# Autodesk Inventor assembly: GearV1
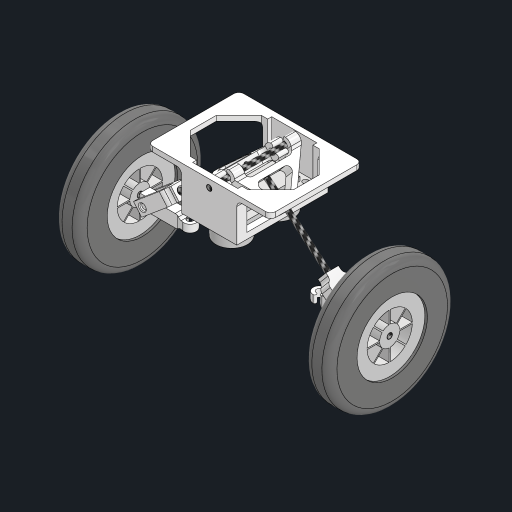
[picture p0: Inventor's stored thumbnail of the model, 512x512]
Saved by Autodesk Inventor 2023 (Build 270158000, 158)
## iProperties
Created: 2022-06-24
Part Number: GearV1
Document SubType Name: Assembly
Designer: legot
Author: legot
## Documents named in this file (11)
- C:\Users\legot\Documents\Inventor\HIKOSAPO\Gear\GearV1.iam
- C:\Users\legot\Documents\Inventor\HIKOSAPO\Ultrasonic_holderV4.ipt
- C:\Users\legot\Documents\Inventor\HIKOSAPO\Gear\Holder's Shaft.ipt
- C:\Users\legot\Documents\Inventor\HIKOSAPO\Gear\GearBase.ipt
- C:\Users\legot\Documents\Inventor\HIKOSAPO\UltrasonicSensor.ipt
- C:\Users\legot\Documents\Inventor\HIKOSAPO\Gear\gear_rod.ipt
- C:\Users\legot\Documents\Inventor\HIKOSAPO\Gear\gear_connecotr1.ipt
- C:\Users\legot\Documents\Inventor\HIKOSAPO\Gear\gear_connector2.ipt
- C:\Users\legot\Documents\Inventor\HIKOSAPO\Gear\gear_shaft1.ipt
- C:\Users\legot\Documents\Inventor\HIKOSAPO\Gear\Tire_Φ50.ipt
- C:\Users\legot\Documents\Inventor\HIKOSAPO\Gear\Wheel_Φ50.ipt
## Components (17 placed, 10 different names)
1. Ultrasonic_holderV4:1 — 挿入:4, 挿入:5, 角度:2, 挿入:14, 挿入:15, 挿入:16, 角度:3
2. Holder's Shaft:1 — 挿入:14
3. GearBase:1 — 挿入:6, 挿入:16, 角度:3
4. GearBase:2 — 挿入:7, 角度:2, 挿入:15
5. UltrasonicSensor:1 — 挿入:4, 挿入:5
6. gear_rod:1 — 挿入:6, 挿入:8
7. gear_rod:2 — 挿入:7, 挿入:9
8. gear_connecotr1:1 — メイト:1, メイト:4, フラッシュ:1, 挿入:10
9. gear_connecotr1:2 — メイト:2, メイト:3, フラッシュ:1, 挿入:11
10. gear_connector2:1 — 挿入:8, メイト:1, メイト:4
11. gear_connector2:2 — 挿入:9, メイト:2, メイト:3
12. gear_shaft1:1 — 挿入:11, 挿入:18
13. gear_shaft1:2 — 挿入:10, 挿入:17
14. Tire_Φ50:1 — フラッシュ:2, メイト:5
15. Tire_Φ50:2 — フラッシュ:3, メイト:6
16. Wheel_Φ50:1 — フラッシュ:2, メイト:5, 挿入:17
17. Wheel_Φ50:2 — フラッシュ:3, 挿入:18, メイト:6
## Relationships (24: Insert 13, Mate 6, Flush 3, Angle 2)
- 挿入:4 [Insert]: Ultrasonic_holderV4:1 ↔ UltrasonicSensor:1
- 挿入:5 [Insert]: Ultrasonic_holderV4:1 ↔ UltrasonicSensor:1
- 挿入:6 [Insert]: GearBase:1 ↔ gear_rod:1
- 挿入:7 [Insert]: GearBase:2 ↔ gear_rod:2
- 角度:2 [Angle] (-45 deg): Ultrasonic_holderV4:1 ↔ GearBase:2
- 挿入:8 [Insert]: gear_rod:1 ↔ gear_connector2:1
- 挿入:9 [Insert]: gear_rod:2 ↔ gear_connector2:2
- メイト:1 [Mate]: gear_connecotr1:1 ↔ gear_connector2:1
- メイト:2 [Mate]: gear_connecotr1:2 ↔ gear_connector2:2
- メイト:3 [Mate]: gear_connecotr1:2 ↔ gear_connector2:2
- メイト:4 [Mate]: gear_connecotr1:1 ↔ gear_connector2:1
- フラッシュ:1 [Flush]: gear_connecotr1:1 ↔ gear_connecotr1:2
- 挿入:10 [Insert] (-10 mm): gear_connecotr1:1 ↔ gear_shaft1:2
- 挿入:11 [Insert] (-10 mm): gear_connecotr1:2 ↔ gear_shaft1:1
- フラッシュ:2 [Flush]: Tire_Φ50:1 ↔ Wheel_Φ50:1
- フラッシュ:3 [Flush]: Tire_Φ50:2 ↔ Wheel_Φ50:2
- 挿入:14 [Insert]: Ultrasonic_holderV4:1 ↔ Holder's Shaft:1
- 挿入:15 [Insert]: Ultrasonic_holderV4:1 ↔ GearBase:2
- 挿入:16 [Insert]: Ultrasonic_holderV4:1 ↔ GearBase:1
- 角度:3 [Angle] (0 deg): Ultrasonic_holderV4:1 ↔ GearBase:1
- メイト:5 [Mate]: Tire_Φ50:1 ↔ Wheel_Φ50:1
- 挿入:17 [Insert]: gear_shaft1:2 ↔ Wheel_Φ50:1
- 挿入:18 [Insert]: gear_shaft1:1 ↔ Wheel_Φ50:2
- メイト:6 [Mate]: Tire_Φ50:2 ↔ Wheel_Φ50:2
